# Autodesk Inventor assembly: aos5
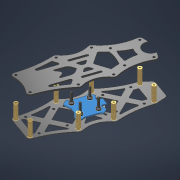
[picture p0: Inventor's stored thumbnail of the model, 180x180]
Saved by Autodesk Inventor 2022 (Build 260153000, 153)
## iProperties
Created: 2022-07-20
Part Number: aos5
Document SubType Name: Assembly
Designer: ancher
Author: ancher
## Documents named in this file (7)
- E:\RC\print_3d\aos5\aos5.iam
- E:\RC\print_3d\aos5\bottom_plate.ipt
- E:\RC\print_3d\aos5\top_plate.ipt
- E:\RC\print_3d\aos5\standoff.ipt
- E:\RC\print_3d\inventor\ContentCenterFiles\en-US\ISO 7380-1\ISO 7380-1 - M3 x 6.ipt
- E:\RC\print_3d\aos5\esc.iam
- E:\RC\print_3d\inventor\ContentCenterFiles\en-US\ISO 7380-1\ISO 7380-1 - M3 x 20.ipt
## Components (23 placed, 6 different names)
1. bottom_plate:1 — Mate:1, Mate:2, Mate:3, Mate:4, Mate:5, Mate:6, Mate:7, Mate:8, Mate:9, Mate:11, Mate:12, Mate:13, Mate:14, Mate:15, Mate:16, Mate:17, Mate:18, Mate:19, Mate:21, Mate:23, Mate:25, Mate:27, Mate:29, Mate:31, Mate:33, Mate:35, Mate:36, Mate:37, Mate:38, Insert:1, Insert:2, Insert:3, Insert:4
2. top_plate:1 — Mate:1, Mate:2
3. standoff:1 — Mate:3, Mate:11, Mate:22
4. standoff:2 — Mate:4, Mate:13, Mate:24
5. standoff:3 — Mate:5, Mate:17, Mate:26
6. standoff:4 — Mate:6, Mate:19, Mate:28
7. standoff:5 — Mate:7, Mate:18, Mate:30
8. standoff:6 — Mate:8, Mate:16, Mate:32
9. standoff:7 — Mate:9, Mate:15, Mate:34
10. standoff:8 — Mate:12, Mate:14, Mate:20
11. ISO 7380-1 M3 x 6:1 — Mate:20, Mate:21
12. ISO 7380-1 M3 x 6:2 — Mate:22, Mate:23
13. ISO 7380-1 M3 x 6:3 — Mate:24, Mate:25
14. ISO 7380-1 M3 x 6:4 — Mate:26, Mate:27
15. ISO 7380-1 M3 x 6:5 — Mate:28, Mate:29
16. ISO 7380-1 M3 x 6:6 — Mate:30, Mate:31
17. ISO 7380-1 M3 x 6:7 — Mate:32, Mate:33
18. ISO 7380-1 M3 x 6:8 — Mate:34, Mate:35
19. esc:1 [sub-assembly] — Mate:36, Mate:37, Mate:38
20. ISO 7380-1 M3 x 20:1 — Insert:1
21. ISO 7380-1 M3 x 20:2 — Insert:2
22. ISO 7380-1 M3 x 20:3 — Insert:3
23. ISO 7380-1 M3 x 20:4 — Insert:4
## Relationships (41: Mate 37, Insert 4)
- Mate:1: bottom_plate:1 ↔ top_plate:1
- Mate:2: bottom_plate:1 ↔ top_plate:1
- Mate:3: bottom_plate:1 ↔ standoff:1
- Mate:4: bottom_plate:1 ↔ standoff:2
- Mate:5: bottom_plate:1 ↔ standoff:3
- Mate:6: bottom_plate:1 ↔ standoff:4
- Mate:7: bottom_plate:1 ↔ standoff:5
- Mate:8: bottom_plate:1 ↔ standoff:6
- Mate:9: bottom_plate:1 ↔ standoff:7
- Mate:11: bottom_plate:1 ↔ standoff:1
- Mate:12: bottom_plate:1 ↔ standoff:8
- Mate:13: bottom_plate:1 ↔ standoff:2
- Mate:14: bottom_plate:1 ↔ standoff:8
- Mate:15: bottom_plate:1 ↔ standoff:7
- Mate:16: bottom_plate:1 ↔ standoff:6
- Mate:17: bottom_plate:1 ↔ standoff:3
- Mate:18: bottom_plate:1 ↔ standoff:5
- Mate:19: bottom_plate:1 ↔ standoff:4
- Mate:20: standoff:8 ↔ ISO 7380-1 M3 x 6:1
- Mate:21: bottom_plate:1 ↔ ISO 7380-1 M3 x 6:1
- Mate:22: standoff:1 ↔ ISO 7380-1 M3 x 6:2
- Mate:23: bottom_plate:1 ↔ ISO 7380-1 M3 x 6:2
- Mate:24: standoff:2 ↔ ISO 7380-1 M3 x 6:3
- Mate:25: bottom_plate:1 ↔ ISO 7380-1 M3 x 6:3
- Mate:26: standoff:3 ↔ ISO 7380-1 M3 x 6:4
- Mate:27: bottom_plate:1 ↔ ISO 7380-1 M3 x 6:4
- Mate:28: standoff:4 ↔ ISO 7380-1 M3 x 6:5
- Mate:29: bottom_plate:1 ↔ ISO 7380-1 M3 x 6:5
- Mate:30: standoff:5 ↔ ISO 7380-1 M3 x 6:6
- Mate:31: bottom_plate:1 ↔ ISO 7380-1 M3 x 6:6
- Mate:32: standoff:6 ↔ ISO 7380-1 M3 x 6:7
- Mate:33: bottom_plate:1 ↔ ISO 7380-1 M3 x 6:7
- Mate:34: standoff:7 ↔ ISO 7380-1 M3 x 6:8
- Mate:35: bottom_plate:1 ↔ ISO 7380-1 M3 x 6:8
- Mate:36: bottom_plate:1 ↔ esc:1
- Mate:37: bottom_plate:1 ↔ esc:1
- Mate:38: bottom_plate:1 ↔ esc:1
- Insert:1: bottom_plate:1 ↔ ISO 7380-1 M3 x 20:1
- Insert:2: bottom_plate:1 ↔ ISO 7380-1 M3 x 20:2
- Insert:3: bottom_plate:1 ↔ ISO 7380-1 M3 x 20:3
- Insert:4: bottom_plate:1 ↔ ISO 7380-1 M3 x 20:4
